# Autodesk Inventor assembly: Left Claw
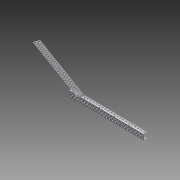
[picture p0: Inventor's stored thumbnail of the model, 180x180]
Saved by Autodesk Inventor 2015 (Build 190159000, 159)
## iProperties
Created: 2016-12-15
Part Number: Left Claw
Document SubType Name: Assembly
Designer: L
Author: L
## Documents named in this file (5)
- C:\Users\L\Google Drive\Engineering Notebook - Leo Wang\StarStuckProject\Starstruck\Prototypes\Left Claw.iam
- C:\Users\L\Google Drive\StarStuckProject\Starstruck\Imported Components\C- Channel 1x2x1x25 2.0\C- Channel 1x2x1x25 2.0.ipt
- C:\Users\L\Google Drive\StarStuckProject\Starstruck\Imported Components\Angle 2x2x25\Angle 2x2x25 Cut.ipt
- C:\Users\L\Google Drive\StarStuckProject\Starstruck\Imported Components\Large Screw .500In\Large Screw .500In.ipt
- C:\Users\L\Google Drive\StarStuckProject\Starstruck\Imported Components\Regular Nut\Regular Nut.ipt
## Components (6 placed, 4 different names)
1. C- Channel 1x2x1x25 2.0:1 — Tangent:1, Tangent:4, Tangent:5, Mate:3, Mate:4, Mate:5, Tangent:8
2. Angle 2x2x25 Cut:1 — Mate:1, Mate:2, Tangent:2, Tangent:3, Mate:3, Tangent:9, Tangent:10
3. Large Screw .500In:1 — Mate:1, Tangent:3, Tangent:4, Tangent:6, Tangent:8, Tangent:9, Tangent:10
4. Large Screw .500In:2 — Mate:2, Tangent:1, Tangent:2, Tangent:5, Tangent:7
5. Regular Nut:1 — Mate:4, Tangent:6
6. Regular Nut:2 — Mate:5, Tangent:7
## Relationships (15: Tangent 10, Mate 5)
- Mate:1: Angle 2x2x25 Cut:1 ↔ Large Screw .500In:1
- Mate:2: Angle 2x2x25 Cut:1 ↔ Large Screw .500In:2
- Tangent:1: C- Channel 1x2x1x25 2.0:1 ↔ Large Screw .500In:2
- Tangent:2: Angle 2x2x25 Cut:1 ↔ Large Screw .500In:2
- Tangent:3: Angle 2x2x25 Cut:1 ↔ Large Screw .500In:1
- Tangent:4: C- Channel 1x2x1x25 2.0:1 ↔ Large Screw .500In:1
- Tangent:5: C- Channel 1x2x1x25 2.0:1 ↔ Large Screw .500In:2
- Mate:3: C- Channel 1x2x1x25 2.0:1 ↔ Angle 2x2x25 Cut:1
- Mate:4: C- Channel 1x2x1x25 2.0:1 ↔ Regular Nut:1
- Tangent:6: Large Screw .500In:1 ↔ Regular Nut:1
- Mate:5: C- Channel 1x2x1x25 2.0:1 ↔ Regular Nut:2
- Tangent:7: Large Screw .500In:2 ↔ Regular Nut:2
- Tangent:8: C- Channel 1x2x1x25 2.0:1 ↔ Large Screw .500In:1
- Tangent:9: Angle 2x2x25 Cut:1 ↔ Large Screw .500In:1
- Tangent:10: Angle 2x2x25 Cut:1 ↔ Large Screw .500In:1
